# Autodesk Inventor assembly: 2100_Tx_Coil_Assm_V1
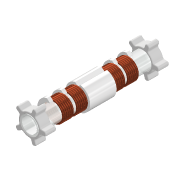
[picture p0: Inventor's stored thumbnail of the model, 180x180]
Saved by Autodesk Inventor 2021 (Build 250183000, 183)
## iProperties
Created: 2022-06-20
Part Number: 2100_Tx_Coil_Assm_V1
Document SubType Name: Assembly
Designer: Eli
Author: Eli
## Documents named in this file (6)
- C:\Users\Eli\Documents\GitHub\MPS\Inventor Parts\MPSV2\2xxx Coil Formers and Parts\21xx Tx Coil\210x Tx Coil Solenoid Former\2100_Tx_Coil_Assm_V1.iam
- C:\Users\Eli\Documents\GitHub\MPS\Inventor Parts\MPSV2\2xxx Coil Formers and Parts\21xx Tx Coil\210x Tx Coil Solenoid Former\2100_Tx_Coil_Former_MPSv2_v4.ipt
- C:\Users\Eli\Documents\GitHub\MPS\Inventor Parts\MPSV2\2xxx Coil Formers and Parts\21xx Tx Coil\210x Tx Coil Solenoid Former\2101_Tx_Coil_Spacer_v1.ipt
- C:\Users\Eli\Documents\GitHub\MPS\Inventor Parts\MPSV2\2xxx Coil Formers and Parts\21xx Tx Coil\210x Tx Coil Solenoid Former\21xx_WireLoop_2,1mm_Inner.ipt
- C:\Users\Eli\Documents\GitHub\MPS\Inventor Parts\MPSV2\2xxx Coil Formers and Parts\21xx Tx Coil\210x Tx Coil Solenoid Former\2101b_Tx_Coil_Spacer_short_v1.ipt
- C:\Users\Eli\Documents\GitHub\MPS\Inventor Parts\MPSV2\2xxx Coil Formers and Parts\21xx Tx Coil\210x Tx Coil Solenoid Former\2102_Tx_Coil_Fins_V1.ipt
## Components (13 placed, 5 different names)
1. 2100_Tx_Coil_Former_MPSv2_v4:1 — Rigid:1, Mate:1, Mate:3, Mate:4, Mate:8, Mate:9, Mate:10, Mate:11, Flush:5, Mate:12, Flush:6, Mate:13, Mate:14, Mate:15
2. 2101_Tx_Coil_Spacer_v1:1 — Flush:1, Flush:2, Flush:3, Mate:2, Mate:7, Tangent:2
3. 2101_Tx_Coil_Spacer_v1:2 — Rigid:1
4. 21xx_WireLoop_2,1mm_Inner:1 — Mate:1, Flush:3
5. 2101b_Tx_Coil_Spacer_short_v1:1 — Mate:2, Mate:3, Mate:5
6. 2101b_Tx_Coil_Spacer_short_v1:2 — Mate:4, Mate:5, Tangent:1
7. 2101b_Tx_Coil_Spacer_short_v1:3 — Mate:9
8. 2101b_Tx_Coil_Spacer_short_v1:4 — Mate:7, Mate:8, Flush:4
9. 21xx_WireLoop_2,1mm_Inner:2 — Flush:4, Mate:10
10. 2102_Tx_Coil_Fins_V1:1 — Mate:11, Flush:5, Flush:7
11. 2102_Tx_Coil_Fins_V1:2 — Mate:12, Flush:6, Flush:7
12. 21xx_WireLoop_2,1mm_Inner:3 — Mate:14, Tangent:2, Mate:15
13. 21xx_WireLoop_2,1mm_Inner:4 — Mate:13, Tangent:1
## Relationships (25: Mate 15, Flush 7, Tangent 2, WeldJoint 1)
- Flush:1: 2101_Tx_Coil_Spacer_v1:1
- Flush:2: 2101_Tx_Coil_Spacer_v1:1
- Rigid:1 [WeldJoint]: 2100_Tx_Coil_Former_MPSv2_v4:1 ↔ 2101_Tx_Coil_Spacer_v1:2
- Mate:1: 2100_Tx_Coil_Former_MPSv2_v4:1 ↔ 21xx_WireLoop_2,1mm_Inner:1
- Flush:3 (-0.75 mm): 2101_Tx_Coil_Spacer_v1:1 ↔ 21xx_WireLoop_2,1mm_Inner:1
- Mate:2 (12 mm): 2101_Tx_Coil_Spacer_v1:1 ↔ 2101b_Tx_Coil_Spacer_short_v1:1
- Mate:3: 2100_Tx_Coil_Former_MPSv2_v4:1 ↔ 2101b_Tx_Coil_Spacer_short_v1:1
- Mate:4: 2100_Tx_Coil_Former_MPSv2_v4:1 ↔ 2101b_Tx_Coil_Spacer_short_v1:2
- Mate:5 (12 mm): 2101b_Tx_Coil_Spacer_short_v1:1 ↔ 2101b_Tx_Coil_Spacer_short_v1:2
- [Mate] (12 mm): 2101b_Tx_Coil_Spacer_short_v1:3 ↔ 2101b_Tx_Coil_Spacer_short_v1:4
- Mate:7 (12 mm): 2101_Tx_Coil_Spacer_v1:1 ↔ 2101b_Tx_Coil_Spacer_short_v1:4
- Mate:8: 2100_Tx_Coil_Former_MPSv2_v4:1 ↔ 2101b_Tx_Coil_Spacer_short_v1:4
- Mate:9: 2100_Tx_Coil_Former_MPSv2_v4:1 ↔ 2101b_Tx_Coil_Spacer_short_v1:3
- Flush:4 (-0.75 mm): 2101b_Tx_Coil_Spacer_short_v1:4 ↔ 21xx_WireLoop_2,1mm_Inner:2
- Mate:10: 2100_Tx_Coil_Former_MPSv2_v4:1 ↔ 21xx_WireLoop_2,1mm_Inner:2
- Mate:11: 2100_Tx_Coil_Former_MPSv2_v4:1 ↔ 2102_Tx_Coil_Fins_V1:1
- Flush:5: 2100_Tx_Coil_Former_MPSv2_v4:1 ↔ 2102_Tx_Coil_Fins_V1:1
- Mate:12: 2100_Tx_Coil_Former_MPSv2_v4:1 ↔ 2102_Tx_Coil_Fins_V1:2
- Flush:6: 2100_Tx_Coil_Former_MPSv2_v4:1 ↔ 2102_Tx_Coil_Fins_V1:2
- Flush:7: 2102_Tx_Coil_Fins_V1:1 ↔ 2102_Tx_Coil_Fins_V1:2
- Mate:13: 2100_Tx_Coil_Former_MPSv2_v4:1 ↔ 21xx_WireLoop_2,1mm_Inner:4
- Mate:14: 2100_Tx_Coil_Former_MPSv2_v4:1 ↔ 21xx_WireLoop_2,1mm_Inner:3
- Tangent:1: 2101b_Tx_Coil_Spacer_short_v1:2 ↔ 21xx_WireLoop_2,1mm_Inner:4
- Tangent:2: 2101_Tx_Coil_Spacer_v1:1 ↔ 21xx_WireLoop_2,1mm_Inner:3
- Mate:15: 2100_Tx_Coil_Former_MPSv2_v4:1 ↔ 21xx_WireLoop_2,1mm_Inner:3
## Named parameters: d11_d10 = 12 mm
